# Autodesk Inventor assembly: Pancake_Reverse Assy_4 Lanes
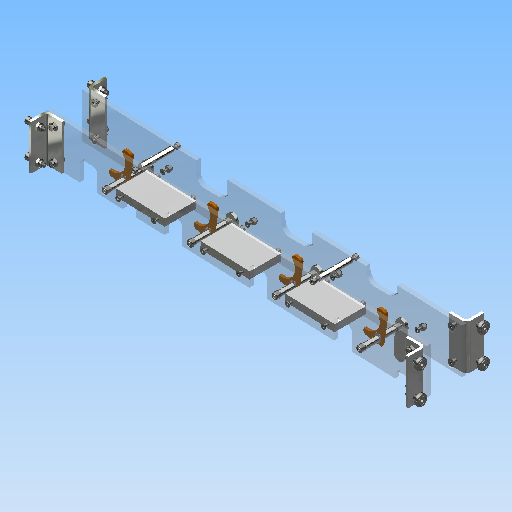
[picture p0: Inventor's stored thumbnail of the model, 512x512]
Saved by Autodesk Inventor 2018.1 (Build 221171000, 171)
## iProperties
Created: 2019-02-11
Part Number: Pancake_Reverse Assy_4 Lanes
Document SubType Name: Assembly
Designer: James
Author: James
## Documents named in this file (19)
- C:\Users\admin\Desktop\Ball Sorting Machine\Ball-Sorting-Machine\Pancake Sort\Pancake - 4 Lanes\Pancake_Reverse Assy_4 Lanes.iam
- C:\Users\admin\Desktop\Ball Sorting Machine\Ball-Sorting-Machine\Timing Gate\Nyloc Nut - M4.ipt
- C:\Users\admin\Desktop\Ball Sorting Machine\Ball-Sorting-Machine\Timing Gate\Socket Cap Screw - Standard - (A2) - M4 x 16.ipt
- C:\Users\admin\Desktop\Ball Sorting Machine\Ball-Sorting-Machine\Pancake Sort\Pancake_Angle Bracket.ipt
- C:\Users\admin\Desktop\Ball Sorting Machine\Ball-Sorting-Machine\Selection Sort\Socket Csk Screw - (A2) - M4 x  12.ipt
- C:\Users\admin\Desktop\Ball Sorting Machine\Ball-Sorting-Machine\Pancake Sort\Pancake_Connector.ipt
- C:\Users\admin\Desktop\Ball Sorting Machine\Ball-Sorting-Machine\Pancake Sort\Socket Cap Screw - Standard - (A2) - M3 x 12.ipt
- C:\Users\admin\Desktop\Ball Sorting Machine\Ball-Sorting-Machine\Pancake Sort\Pancake_Bearing.ipt
- C:\Users\admin\Desktop\Ball Sorting Machine\Ball-Sorting-Machine\Pancake Sort\Pancake_Reverse Shaft.ipt
- C:\Users\admin\Desktop\Ball Sorting Machine\Ball-Sorting-Machine\Pancake Sort\Pancake_Reverse Lever.ipt
- C:\Users\admin\Desktop\Ball Sorting Machine\Ball-Sorting-Machine\Timing Gate\BS 3673 - 6mm External Circlip.ipt
- C:\Users\admin\Desktop\Ball Sorting Machine\Ball-Sorting-Machine\Pancake Sort\Pancake_Reverse Weight.ipt
- C:\Users\admin\Desktop\Ball Sorting Machine\Ball-Sorting-Machine\Selection Sort\Locknut - M3.ipt
- C:\Users\admin\Desktop\Ball Sorting Machine\Ball-Sorting-Machine\Pancake Sort\Socket Csk Screw - (A2) - M3 x  10.ipt
- C:\Users\admin\Desktop\Ball Sorting Machine\Ball-Sorting-Machine\Pancake Sort\Pancake_Floor Piece.ipt
- C:\Users\admin\Desktop\Ball Sorting Machine\Ball-Sorting-Machine\Pancake Sort\Pancake - 4 Lanes\Pancake_Reverse Backboard 2_4 Lanes.ipt
- C:\Users\admin\Desktop\Ball Sorting Machine\Ball-Sorting-Machine\Pancake Sort\Pancake - 4 Lanes\Pancake_Reverse Backboard_4 Lanes.ipt
- C:\Users\admin\Desktop\Ball Sorting Machine\Ball-Sorting-Machine\Pancake Sort\FWSRS-D12-V4.5-E2.5-T3_.ipt
- C:\Users\admin\Desktop\Ball Sorting Machine\Ball-Sorting-Machine\Pancake Sort\Socket Csk Screw - (A2) - M4 x  16.ipt
## Components (95 placed, 18 different names)
1. Pancake_Reverse Backboard 2_4 Lanes:1 — Mate:104, Mate:105, Mate:106, Flush:36, Mate:115, Flush:37, Mate:118, Mate:119, Mate:132, Tangent:2, Mate:138, Tangent:3, Mate:140, Mate:141, Tangent:4, Tangent:5, Mate:144, Flush:104, Flush:105, Mate:176, Mate:177, Mate:179, Mate:180, Mate:181, Mate:182, Mate:183, Mate:188, Mate:189, Flush:110, Flush:111, Mate:192, Mate:200, Mate:201, Mate:202, Mate:203, Mate:204, Tangent:15, Tangent:16
2. Pancake_Angle Bracket:3 — Mate:104, Mate:105, Mate:106, Flush:36, Mate:124, Mate:125, Mate:126, Mate:127, Mate:134, Mate:139
3. Pancake_Angle Bracket:4 — Mate:115, Flush:37, Mate:118, Mate:119, Mate:131, Mate:142, Mate:143, Mate:209, Mate:210, Mate:215
4. Pancake_Reverse Backboard_4 Lanes:1 — Mate:144, Flush:104, Flush:105, Mate:155, Mate:156, Mate:157, Mate:158, Mate:159, Tangent:6, Tangent:7, Mate:170, Mate:171, Mate:173, Mate:174, Tangent:8, Tangent:9, Mate:175, Mate:178, Mate:184, Mate:185, Mate:186, Mate:187, Mate:190, Flush:112, Flush:113, Mate:197, Tangent:12, Mate:198, Mate:205, Mate:206, Mate:207, Mate:208, Tangent:13, Tangent:14
5. Pancake_Angle Bracket:5 — Mate:155, Mate:156, Mate:157
6. Pancake_Angle Bracket:6 — Mate:170, Mate:171, Mate:175, Mate:216, Mate:217
7. Pancake_Connector:1 — Mate:176, Mate:177, Mate:178
8. Pancake_Connector:2 — Mate:179, Mate:180
9. Socket Csk Screw - (A2) - M4 x  16:5 — Mate:210, Mate:211, Tangent:17, Mate:218
10. FWSRS-D12-V4.5-E2.5-T3.0:5 — Mate:209, Mate:211, Tangent:17, Flush:116, Flush:118
11. Socket Csk Screw - (A2) - M4 x  16:6 — Mate:215, Mate:219
12. FWSRS-D12-V4.5-E2.5-T3.0:6 — Flush:116
13. Socket Csk Screw - (A2) - M4 x  16:7 — Mate:216, Mate:221
14. FWSRS-D12-V4.5-E2.5-T3.0:7 — Flush:117
15. Socket Csk Screw - (A2) - M4 x  16:8 — Mate:217, Mate:220
16. FWSRS-D12-V4.5-E2.5-T3.0:8 — Flush:117, Flush:118
17. Socket Cap Screw - Standard - (A2) - M4 x 16:11 — Flush:98, Mate:125, Mate:126
18. Nyloc Nut - M4:37 — Flush:99, Mate:127
19. Socket Cap Screw - Standard - (A2) - M4 x 16:12 — Flush:98, Mate:124
20. Nyloc Nut - M4:38 — Flush:99
21. Nyloc Nut - M4:39 — Flush:101, Mate:131, Mate:218
22. Nyloc Nut - M4:40 — Flush:101, Mate:219
23. Socket Csk Screw - (A2) - M4 x  12:1 — Mate:132, Tangent:2, Mate:133
24. Nyloc Nut - M4:41 — Mate:133, Mate:134
25. Socket Csk Screw - (A2) - M4 x  12:2 — Mate:138, Tangent:3
26. Nyloc Nut - M4:42 — Mate:139
27. Socket Csk Screw - (A2) - M4 x  12:3 — Mate:141, Tangent:4
28. Nyloc Nut - M4:43 — Mate:142
29. Socket Csk Screw - (A2) - M4 x  12:4 — Mate:140, Tangent:5
30. Nyloc Nut - M4:44 — Mate:143
31. Socket Cap Screw - Standard - (A2) - M4 x 16:15
32. Nyloc Nut - M4:45
33. Socket Cap Screw - Standard - (A2) - M4 x 16:16
34. Nyloc Nut - M4:46
35. Socket Csk Screw - (A2) - M4 x  12:5 — Mate:158, Tangent:6
36. Nyloc Nut - M4:47
37. Socket Csk Screw - (A2) - M4 x  12:6 — Mate:159, Tangent:7
38. Nyloc Nut - M4:48
39. Nyloc Nut - M4:49 — Mate:220
40. Nyloc Nut - M4:50 — Mate:221
41. Socket Csk Screw - (A2) - M4 x  12:7 — Mate:173, Tangent:8
42. Nyloc Nut - M4:51
43. Socket Csk Screw - (A2) - M4 x  12:8 — Mate:174, Tangent:9
44. Nyloc Nut - M4:52
45. Socket Cap Screw - Standard - (A2) - M3 x 12:1 — Mate:181, Mate:182
46. Socket Cap Screw - Standard - (A2) - M3 x 12:2 — Mate:183, Mate:188
47. Socket Cap Screw - Standard - (A2) - M3 x 12:3 — Mate:184, Mate:187
48. Socket Cap Screw - Standard - (A2) - M3 x 12:4 — Mate:185, Mate:186
49. BS 3673 - 6mm External Circlip:1 — Mate:194, Mate:195, Angle:1
50. Pancake_Reverse Lever:1 — Mate:193, Flush:114, Angle:1, Angle:2
51. Pancake_Reverse Shaft:1 — Mate:191, Mate:192, Mate:193, Flush:114, Mate:194, Mate:195, Mate:196, Flush:115
52. Pancake_Bearing:1 — Mate:189, Flush:110, Flush:111, Mate:191
53. Pancake_Reverse Weight:1 — Mate:196, Flush:115, Angle:2
54. Pancake_Bearing:2 — Mate:190, Flush:112, Flush:113
55. BS 3673 - 6mm External Circlip:2
56. Pancake_Reverse Lever:2
57. Pancake_Reverse Shaft:2
58. Pancake_Bearing:3
59. Pancake_Reverse Weight:2
60. Pancake_Bearing:4
61. BS 3673 - 6mm External Circlip:3
62. Pancake_Reverse Lever:3
63. Pancake_Reverse Shaft:3
64. Pancake_Bearing:5
65. Pancake_Reverse Weight:3
66. Pancake_Bearing:6
67. BS 3673 - 6mm External Circlip:4
68. Pancake_Reverse Lever:4
69. Pancake_Reverse Shaft:4
70. Pancake_Bearing:7
71. Pancake_Reverse Weight:4
72. Pancake_Bearing:8
73. Socket Csk Screw - (A2) - M3 x  10:1 — Mate:197, Tangent:12, Mate:199
74. Locknut - M3:1 — Mate:198, Mate:199
75. Socket Csk Screw - (A2) - M3 x  10:2
76. Locknut - M3:2
77. Socket Csk Screw - (A2) - M3 x  10:3
78. Locknut - M3:3
79. Socket Csk Screw - (A2) - M3 x  10:4
80. Locknut - M3:4
81. Pancake_Floor Piece:1 — Mate:200, Mate:201, Mate:202, Mate:207, Mate:208
82. Socket Csk Screw - (A2) - M3 x  10:9 — Mate:205, Tangent:13
83. Socket Csk Screw - (A2) - M3 x  10:8 — Mate:203, Tangent:15
84. Socket Csk Screw - (A2) - M3 x  10:7 — Mate:206, Tangent:14
85. Socket Csk Screw - (A2) - M3 x  10:6 — Mate:204, Tangent:16
86. Pancake_Floor Piece:2
87. Socket Csk Screw - (A2) - M3 x  10:10
88. Socket Csk Screw - (A2) - M3 x  10:11
89. Socket Csk Screw - (A2) - M3 x  10:12
90. Socket Csk Screw - (A2) - M3 x  10:13
91. Pancake_Floor Piece:3
92. Socket Csk Screw - (A2) - M3 x  10:14
93. Socket Csk Screw - (A2) - M3 x  10:15
94. Socket Csk Screw - (A2) - M3 x  10:16
95. Socket Csk Screw - (A2) - M3 x  10:17
## Component patterns: (4 elements, first: BS 3673 - 6mm External Circlip:1 + Pancake_Reverse Lever:1 + Pancake_Reverse Shaft:1 + Pancake_Bearing:1 + Pancake_Reverse Weight:1 + Pancake_Bearing:2), (4 elements, first: Socket Csk Screw - (A2) - M3 x  10:1 + Locknut - M3:1), (3 elements, first: Pancake_Floor Piece:1 + Socket Csk Screw - (A2) - M3 x  10:9 + Socket Csk Screw - (A2) - M3 x  10:8 + Socket Csk Screw - (A2) - M3 x  10:7 + Socket Csk Screw - (A2) - M3 x  10:6)
## Relationships (140: Mate 97, Flush 24, Tangent 17, Angle 2)
- Flush:11 (62.5 mm)
- [Flush]: Pancake_Reverse Backboard 2_4 Lanes:1
- [Flush]: Pancake_Reverse Backboard 2_4 Lanes:1
- [Flush]: Pancake_Reverse Backboard 2_4 Lanes:1
- Mate:104: Pancake_Reverse Backboard 2_4 Lanes:1 ↔ Pancake_Angle Bracket:3
- Mate:105: Pancake_Reverse Backboard 2_4 Lanes:1 ↔ Pancake_Angle Bracket:3
- Mate:106: Pancake_Reverse Backboard 2_4 Lanes:1 ↔ Pancake_Angle Bracket:3
- Flush:36: Pancake_Reverse Backboard 2_4 Lanes:1 ↔ Pancake_Angle Bracket:3
- Mate:115: Pancake_Reverse Backboard 2_4 Lanes:1 ↔ Pancake_Angle Bracket:4
- Flush:37: Pancake_Reverse Backboard 2_4 Lanes:1 ↔ Pancake_Angle Bracket:4
- Mate:118: Pancake_Reverse Backboard 2_4 Lanes:1 ↔ Pancake_Angle Bracket:4
- Mate:119: Pancake_Reverse Backboard 2_4 Lanes:1 ↔ Pancake_Angle Bracket:4
- [Mate]: Socket Cap Screw - Standard - (A2) - M4 x 16:11 ↔ Nyloc Nut - M4:37
- [Mate]: Socket Cap Screw - Standard - (A2) - M4 x 16:12 ↔ Nyloc Nut - M4:38
- Flush:98: Socket Cap Screw - Standard - (A2) - M4 x 16:11 ↔ Socket Cap Screw - Standard - (A2) - M4 x 16:12
- Mate:124: Pancake_Angle Bracket:3 ↔ Socket Cap Screw - Standard - (A2) - M4 x 16:12
- Mate:125: Pancake_Angle Bracket:3 ↔ Socket Cap Screw - Standard - (A2) - M4 x 16:11
- Mate:126 (5 mm): Pancake_Angle Bracket:3 ↔ Socket Cap Screw - Standard - (A2) - M4 x 16:11
- Flush:99: Nyloc Nut - M4:37 ↔ Nyloc Nut - M4:38
- Mate:127: Pancake_Angle Bracket:3 ↔ Nyloc Nut - M4:37
- Flush:101: Nyloc Nut - M4:39 ↔ Nyloc Nut - M4:40
- Mate:131: Pancake_Angle Bracket:4 ↔ Nyloc Nut - M4:39
- Flush:103 (35 mm)
- Mate:132: Pancake_Reverse Backboard 2_4 Lanes:1 ↔ Socket Csk Screw - (A2) - M4 x  12:1
- Tangent:2: Pancake_Reverse Backboard 2_4 Lanes:1 ↔ Socket Csk Screw - (A2) - M4 x  12:1
- Mate:133: Socket Csk Screw - (A2) - M4 x  12:1 ↔ Nyloc Nut - M4:41
- Mate:134: Pancake_Angle Bracket:3 ↔ Nyloc Nut - M4:41
- [Mate]: Socket Csk Screw - (A2) - M4 x  12:2 ↔ Nyloc Nut - M4:42
- [Mate]: Socket Csk Screw - (A2) - M4 x  12:3 ↔ Nyloc Nut - M4:43
- [Mate]: Socket Csk Screw - (A2) - M4 x  12:4 ↔ Nyloc Nut - M4:44
- Mate:138: Pancake_Reverse Backboard 2_4 Lanes:1 ↔ Socket Csk Screw - (A2) - M4 x  12:2
- Tangent:3: Pancake_Reverse Backboard 2_4 Lanes:1 ↔ Socket Csk Screw - (A2) - M4 x  12:2
- Mate:139: Pancake_Angle Bracket:3 ↔ Nyloc Nut - M4:42
- Mate:140: Pancake_Reverse Backboard 2_4 Lanes:1 ↔ Socket Csk Screw - (A2) - M4 x  12:4
- Mate:141: Pancake_Reverse Backboard 2_4 Lanes:1 ↔ Socket Csk Screw - (A2) - M4 x  12:3
- Tangent:4: Pancake_Reverse Backboard 2_4 Lanes:1 ↔ Socket Csk Screw - (A2) - M4 x  12:3
- Tangent:5: Pancake_Reverse Backboard 2_4 Lanes:1 ↔ Socket Csk Screw - (A2) - M4 x  12:4
- Mate:142: Pancake_Angle Bracket:4 ↔ Nyloc Nut - M4:43
- Mate:143: Pancake_Angle Bracket:4 ↔ Nyloc Nut - M4:44
- Mate:144 (35 mm): Pancake_Reverse Backboard 2_4 Lanes:1 ↔ Pancake_Reverse Backboard_4 Lanes:1
- Flush:104: Pancake_Reverse Backboard 2_4 Lanes:1 ↔ Pancake_Reverse Backboard_4 Lanes:1
- Flush:105: Pancake_Reverse Backboard 2_4 Lanes:1 ↔ Pancake_Reverse Backboard_4 Lanes:1
- [Mate]: Socket Cap Screw - Standard - (A2) - M4 x 16:15 ↔ Nyloc Nut - M4:45
- [Mate]: Socket Cap Screw - Standard - (A2) - M4 x 16:16 ↔ Nyloc Nut - M4:46
- [Flush]: Socket Cap Screw - Standard - (A2) - M4 x 16:15 ↔ Socket Cap Screw - Standard - (A2) - M4 x 16:16
- [Mate]: Pancake_Angle Bracket:5 ↔ Socket Cap Screw - Standard - (A2) - M4 x 16:16
- [Mate]: Pancake_Angle Bracket:5 ↔ Socket Cap Screw - Standard - (A2) - M4 x 16:15
- [Mate] (5 mm): Pancake_Angle Bracket:5 ↔ Socket Cap Screw - Standard - (A2) - M4 x 16:15
- [Flush]: Nyloc Nut - M4:45 ↔ Nyloc Nut - M4:46
- [Mate]: Pancake_Angle Bracket:5 ↔ Nyloc Nut - M4:45
- [Mate]: Socket Csk Screw - (A2) - M4 x  12:5 ↔ Nyloc Nut - M4:47
- [Mate]: Pancake_Angle Bracket:5 ↔ Nyloc Nut - M4:47
- [Mate]: Socket Csk Screw - (A2) - M4 x  12:6 ↔ Nyloc Nut - M4:48
- [Mate]: Pancake_Angle Bracket:5 ↔ Nyloc Nut - M4:48
- Mate:155: Pancake_Reverse Backboard_4 Lanes:1 ↔ Pancake_Angle Bracket:5
- Mate:156: Pancake_Reverse Backboard_4 Lanes:1 ↔ Pancake_Angle Bracket:5
- Mate:157: Pancake_Reverse Backboard_4 Lanes:1 ↔ Pancake_Angle Bracket:5
- Mate:158: Pancake_Reverse Backboard_4 Lanes:1 ↔ Socket Csk Screw - (A2) - M4 x  12:5
- Mate:159: Pancake_Reverse Backboard_4 Lanes:1 ↔ Socket Csk Screw - (A2) - M4 x  12:6
- Tangent:6: Pancake_Reverse Backboard_4 Lanes:1 ↔ Socket Csk Screw - (A2) - M4 x  12:5
- Tangent:7: Pancake_Reverse Backboard_4 Lanes:1 ↔ Socket Csk Screw - (A2) - M4 x  12:6
- [Flush]: Nyloc Nut - M4:49 ↔ Nyloc Nut - M4:50
- [Mate]: Pancake_Angle Bracket:6 ↔ Nyloc Nut - M4:49
- [Mate]: Socket Csk Screw - (A2) - M4 x  12:7 ↔ Nyloc Nut - M4:51
- [Mate]: Pancake_Angle Bracket:6 ↔ Nyloc Nut - M4:51
- [Mate]: Socket Csk Screw - (A2) - M4 x  12:8 ↔ Nyloc Nut - M4:52
- [Mate]: Pancake_Angle Bracket:6 ↔ Nyloc Nut - M4:52
- Mate:170: Pancake_Reverse Backboard_4 Lanes:1 ↔ Pancake_Angle Bracket:6
- Mate:171: Pancake_Reverse Backboard_4 Lanes:1 ↔ Pancake_Angle Bracket:6
- Mate:173: Pancake_Reverse Backboard_4 Lanes:1 ↔ Socket Csk Screw - (A2) - M4 x  12:7
- Mate:174: Pancake_Reverse Backboard_4 Lanes:1 ↔ Socket Csk Screw - (A2) - M4 x  12:8
- Tangent:8: Pancake_Reverse Backboard_4 Lanes:1 ↔ Socket Csk Screw - (A2) - M4 x  12:7
- Tangent:9: Pancake_Reverse Backboard_4 Lanes:1 ↔ Socket Csk Screw - (A2) - M4 x  12:8
- Mate:175: Pancake_Reverse Backboard_4 Lanes:1 ↔ Pancake_Angle Bracket:6
- Mate:176: Pancake_Reverse Backboard 2_4 Lanes:1 ↔ Pancake_Connector:1
- Mate:177: Pancake_Reverse Backboard 2_4 Lanes:1 ↔ Pancake_Connector:1
- Mate:178: Pancake_Reverse Backboard_4 Lanes:1 ↔ Pancake_Connector:1
- Mate:179: Pancake_Reverse Backboard 2_4 Lanes:1 ↔ Pancake_Connector:2
- Mate:180: Pancake_Reverse Backboard 2_4 Lanes:1 ↔ Pancake_Connector:2
- Mate:181: Pancake_Reverse Backboard 2_4 Lanes:1 ↔ Socket Cap Screw - Standard - (A2) - M3 x 12:1
- Mate:182: Pancake_Reverse Backboard 2_4 Lanes:1 ↔ Socket Cap Screw - Standard - (A2) - M3 x 12:1
- Mate:183: Pancake_Reverse Backboard 2_4 Lanes:1 ↔ Socket Cap Screw - Standard - (A2) - M3 x 12:2
- Mate:184: Pancake_Reverse Backboard_4 Lanes:1 ↔ Socket Cap Screw - Standard - (A2) - M3 x 12:3
- Mate:185: Pancake_Reverse Backboard_4 Lanes:1 ↔ Socket Cap Screw - Standard - (A2) - M3 x 12:4
- Mate:186: Pancake_Reverse Backboard_4 Lanes:1 ↔ Socket Cap Screw - Standard - (A2) - M3 x 12:4
- Mate:187: Pancake_Reverse Backboard_4 Lanes:1 ↔ Socket Cap Screw - Standard - (A2) - M3 x 12:3
- Mate:188: Pancake_Reverse Backboard 2_4 Lanes:1 ↔ Socket Cap Screw - Standard - (A2) - M3 x 12:2
- Mate:189: Pancake_Reverse Backboard 2_4 Lanes:1 ↔ Pancake_Bearing:1
- Flush:110: Pancake_Reverse Backboard 2_4 Lanes:1 ↔ Pancake_Bearing:1
- Flush:111: Pancake_Reverse Backboard 2_4 Lanes:1 ↔ Pancake_Bearing:1
- Mate:190: Pancake_Reverse Backboard_4 Lanes:1 ↔ Pancake_Bearing:2
- Flush:112: Pancake_Reverse Backboard_4 Lanes:1 ↔ Pancake_Bearing:2
- Flush:113: Pancake_Reverse Backboard_4 Lanes:1 ↔ Pancake_Bearing:2
- Mate:191: Pancake_Reverse Shaft:1 ↔ Pancake_Bearing:1
- Mate:192 (0.5 mm): Pancake_Reverse Backboard 2_4 Lanes:1 ↔ Pancake_Reverse Shaft:1
- Mate:193: Pancake_Reverse Lever:1 ↔ Pancake_Reverse Shaft:1
- Flush:114: Pancake_Reverse Lever:1 ↔ Pancake_Reverse Shaft:1
- Mate:194: BS 3673 - 6mm External Circlip:1 ↔ Pancake_Reverse Shaft:1
- Mate:195: BS 3673 - 6mm External Circlip:1 ↔ Pancake_Reverse Shaft:1
- Angle:1 (0 deg): BS 3673 - 6mm External Circlip:1 ↔ Pancake_Reverse Lever:1
- Mate:196: Pancake_Reverse Shaft:1 ↔ Pancake_Reverse Weight:1
- Flush:115 (-0.5 mm): Pancake_Reverse Shaft:1 ↔ Pancake_Reverse Weight:1
- Angle:2 (5 deg): Pancake_Reverse Lever:1 ↔ Pancake_Reverse Weight:1
- Mate:197: Pancake_Reverse Backboard_4 Lanes:1 ↔ Socket Csk Screw - (A2) - M3 x  10:1
- Tangent:12: Pancake_Reverse Backboard_4 Lanes:1 ↔ Socket Csk Screw - (A2) - M3 x  10:1
- Mate:198: Pancake_Reverse Backboard_4 Lanes:1 ↔ Locknut - M3:1
- Mate:199: Socket Csk Screw - (A2) - M3 x  10:1 ↔ Locknut - M3:1
- Mate:200: Pancake_Reverse Backboard 2_4 Lanes:1 ↔ Pancake_Floor Piece:1
- Mate:201: Pancake_Reverse Backboard 2_4 Lanes:1 ↔ Pancake_Floor Piece:1
- Mate:202: Pancake_Reverse Backboard 2_4 Lanes:1 ↔ Pancake_Floor Piece:1
- Mate:203: Pancake_Reverse Backboard 2_4 Lanes:1 ↔ Socket Csk Screw - (A2) - M3 x  10:8
- Mate:204: Pancake_Reverse Backboard 2_4 Lanes:1 ↔ Socket Csk Screw - (A2) - M3 x  10:6
- Mate:205: Pancake_Reverse Backboard_4 Lanes:1 ↔ Socket Csk Screw - (A2) - M3 x  10:9
- Mate:206: Pancake_Reverse Backboard_4 Lanes:1 ↔ Socket Csk Screw - (A2) - M3 x  10:7
- Mate:207: Pancake_Reverse Backboard_4 Lanes:1 ↔ Pancake_Floor Piece:1
- Mate:208: Pancake_Reverse Backboard_4 Lanes:1 ↔ Pancake_Floor Piece:1
- Tangent:13: Pancake_Reverse Backboard_4 Lanes:1 ↔ Socket Csk Screw - (A2) - M3 x  10:9
- Tangent:14: Pancake_Reverse Backboard_4 Lanes:1 ↔ Socket Csk Screw - (A2) - M3 x  10:7
- Tangent:15: Pancake_Reverse Backboard 2_4 Lanes:1 ↔ Socket Csk Screw - (A2) - M3 x  10:8
- Tangent:16: Pancake_Reverse Backboard 2_4 Lanes:1 ↔ Socket Csk Screw - (A2) - M3 x  10:6
- Mate:209 (5 mm): Pancake_Angle Bracket:4 ↔ FWSRS-D12-V4.5-E2.5-T3.0:5
- Mate:210: Pancake_Angle Bracket:4 ↔ Socket Csk Screw - (A2) - M4 x  16:5
- Mate:211: Socket Csk Screw - (A2) - M4 x  16:5 ↔ FWSRS-D12-V4.5-E2.5-T3.0:5
- Tangent:17: Socket Csk Screw - (A2) - M4 x  16:5 ↔ FWSRS-D12-V4.5-E2.5-T3.0:5
- [Mate]: Socket Csk Screw - (A2) - M4 x  16:6 ↔ FWSRS-D12-V4.5-E2.5-T3.0:6
- [Tangent]: Socket Csk Screw - (A2) - M4 x  16:6 ↔ FWSRS-D12-V4.5-E2.5-T3.0:6
- [Mate]: Socket Csk Screw - (A2) - M4 x  16:7 ↔ FWSRS-D12-V4.5-E2.5-T3.0:7
- [Tangent]: Socket Csk Screw - (A2) - M4 x  16:7 ↔ FWSRS-D12-V4.5-E2.5-T3.0:7
- [Mate]: Socket Csk Screw - (A2) - M4 x  16:8 ↔ FWSRS-D12-V4.5-E2.5-T3.0:8
- [Tangent]: Socket Csk Screw - (A2) - M4 x  16:8 ↔ FWSRS-D12-V4.5-E2.5-T3.0:8
- Flush:116: FWSRS-D12-V4.5-E2.5-T3.0:5 ↔ FWSRS-D12-V4.5-E2.5-T3.0:6
- Mate:215: Pancake_Angle Bracket:4 ↔ Socket Csk Screw - (A2) - M4 x  16:6
- Mate:216: Pancake_Angle Bracket:6 ↔ Socket Csk Screw - (A2) - M4 x  16:7
- Mate:217: Pancake_Angle Bracket:6 ↔ Socket Csk Screw - (A2) - M4 x  16:8
- Flush:117: FWSRS-D12-V4.5-E2.5-T3.0:7 ↔ FWSRS-D12-V4.5-E2.5-T3.0:8
- Flush:118: FWSRS-D12-V4.5-E2.5-T3.0:5 ↔ FWSRS-D12-V4.5-E2.5-T3.0:8
- Mate:218: Socket Csk Screw - (A2) - M4 x  16:5 ↔ Nyloc Nut - M4:39
- Mate:219: Socket Csk Screw - (A2) - M4 x  16:6 ↔ Nyloc Nut - M4:40
- Mate:220: Socket Csk Screw - (A2) - M4 x  16:8 ↔ Nyloc Nut - M4:49
- Mate:221: Socket Csk Screw - (A2) - M4 x  16:7 ↔ Nyloc Nut - M4:50
## Named parameters: d211_d172_d149 = 0 mm, d212_d172_d149 = 0 mm, d253_d251 = 0 mm, d254_d251 = 0 mm, d255_d251 = 0 mm, d268_d251 = 0 mm, d269_d252 = 0 mm, d270_d253_d251 = 0 mm, d271_d258 = 0 mm, d272_d215 = 0 mm, d273_d216 = 0 mm, d274_d217 = 0 mm, d275_d218 = 5 mm, d276_d219 = 0 mm, d277_d220 = 0 mm, d278_d211_d172_d149 = 0 mm, d279_d212_d172_d149 = 0 mm, d287_d251 = 0 mm, d288_d252 = 0 mm, d289_d253_d251 = 0 mm, d290_d258 = 0 mm, d295_d219 = 0 mm, d296_d220 = 0 mm, d389_d387 = 0 mm, d390_d388 = 0 mm, d391_d387 = 0 mm, d392_d388 = 0 mm, d393_d387 = 0 mm, d394_d388 = 0 mm
